# Autodesk Inventor assembly: Assembly_Autofocus_10x_laser_espcam_v1
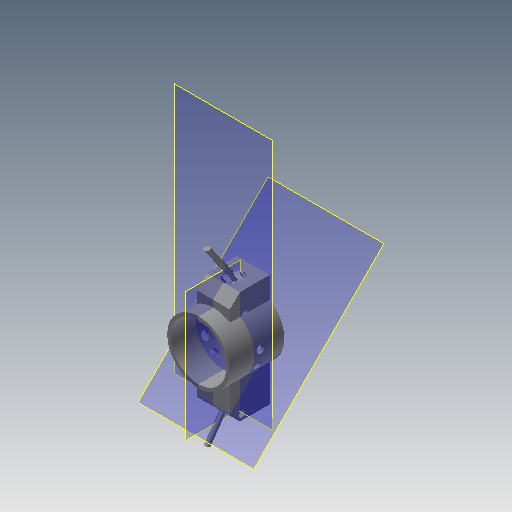
[picture p0: Inventor's stored thumbnail of the model, 512x512]
Saved by Autodesk Inventor 2019.4 (Build 234330000, 330)
## iProperties
Created: 2021-01-19
Part Number: Assembly_Autofocus_10x_laser_espcam_v1
Document SubType Name: Assembly
Designer: diederichbenedict
Author: diederichbenedict
## Documents named in this file (5)
- C:\Users\diederichbenedict\Dropbox\Dokumente\Promotion\PROJECTS\OPENTRONS\INVENTOR\Assembly_Autofocus_10x_laser_espcam_v1.iam
- C:\Users\diederichbenedict\Dropbox\Dokumente\Promotion\PROJECTS\OPENTRONS\INVENTOR\00_Beampath_Autofocus _2.ipt
- C:\Users\diederichbenedict\Dropbox\Dokumente\Promotion\PROJECTS\OPENTRONS\INVENTOR\00_IR_Laserdiode.ipt
- C:\Users\diederichbenedict\Dropbox\Dokumente\Promotion\PROJECTS\OPENTRONS\INVENTOR\13_Opentrons_Autofocus_Objectivering_Laser_Cam.ipt
- C:\Users\diederichbenedict\Dropbox\Dokumente\Promotion\PROJECTS\OPENTRONS\INVENTOR\00_ESP32_Camera_only.ipt
## Components (4 placed, 4 different names)
1. 13_Opentrons_Autofocus_Objectivering_Laser_Cam:1 — Mate:3
2. 00_Beampath_Autofocus _2:1 — Mate:2
3. 00_IR_Laserdiode:1
4. 00_ESP32_Camera_only:1 — Mate:2, Angle:1, Mate:3
## Relationships (5: Mate 3, Flush 1, Angle 1)
- [Mate]: 00_Beampath_Autofocus _2:1 ↔ 00_IR_Laserdiode:1
- [Flush]: 13_Opentrons_Autofocus_Objectivering_Laser_Cam:1 ↔ 00_IR_Laserdiode:1
- Mate:2: 00_Beampath_Autofocus _2:1 ↔ 00_ESP32_Camera_only:1
- Angle:1 (0 deg): 00_ESP32_Camera_only:1
- Mate:3: 13_Opentrons_Autofocus_Objectivering_Laser_Cam:1 ↔ 00_ESP32_Camera_only:1
